# Autodesk Inventor assembly: Cucina
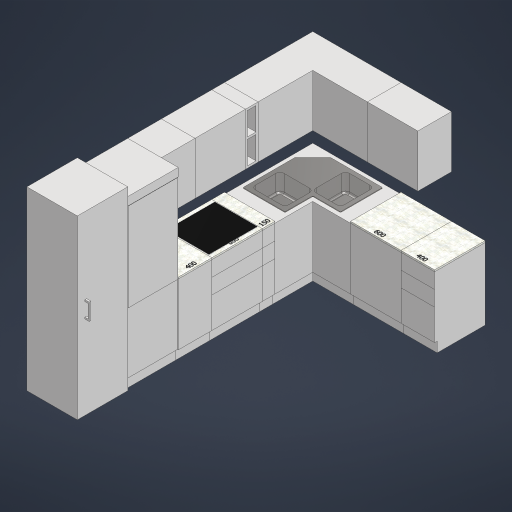
[picture p0: Inventor's stored thumbnail of the model, 512x512]
Saved by Autodesk Inventor 2024.2 (Build 282272000, 272)
## iProperties
Created: 2025-08-27
Part Number: Cucina
Document SubType Name: Assembly
Designer: Luca
Author: Luca
## iProperties of the stored document MemberDocs/xUfgzgntkA0k4y0erJhm34xwdJg
Created: 2025-08-27
Part Number: Cucina
Document SubType Name: Assembly
Designer: Luca
Mass: 4.3593e+06 g
Surface Area: 422535 cm^2
Volume: 4.3593e+06 cm^3
Density: 1 g/cm^3
Author: Luca
## iProperties of the stored document MemberDocs/xWfym0oruPsuzs3vjEgnhmlbwMf
Created: 2025-08-27
Part Number: Cucina
Document SubType Name: Assembly
Designer: Luca
Mass: 4.21038e+06 g
Surface Area: 416936 cm^2
Volume: 4.21038e+06 cm^3
Density: 1 g/cm^3
Author: Luca
## Documents named in this file (10)
- C:\Users\tecnico11\Desktop\Luca\Torre\Cucina.iam
- C:\Users\tecnico11\Desktop\Luca\Torre\Mobile lavandino angolo.ipt
- C:\Users\tecnico11\Desktop\Luca\Torre\Lavandino ad angolo Apell ROAN2IBC.ipt
- C:\Users\tecnico11\Desktop\Luca\Torre\Frigorifero.ipt
- C:\Users\tecnico11\Desktop\Luca\Torre\Mobile cucina.ipt
- C:\Users\tecnico11\Desktop\Luca\Torre\Piano cottura.ipt
- C:\Users\tecnico11\Desktop\Luca\Torre\Pensile.ipt
- C:\Users\tecnico11\Desktop\Luca\Torre\Pensile angolo.ipt
- C:\Users\tecnico11\Desktop\Luca\Torre\Mobile angolo.ipt
- C:\Users\tecnico11\Desktop\Luca\Torre\Mobile lavandino.ipt
## Components (15 placed, 7 different names)
1. Mobile lavandino angolo:1 — Mate:5, Mate:6, Mate:7, Rigid:10, Rigid:13
2. Lavandino ad angolo Apell ROAN2IBC:1
3. Frigorifero:1 — Rigid:11
4. Mobile cucina:1 — Rigid:11
5. Mobile cucina:2 — Rigid:13
6. Mobile cucina:3 — Rigid:10
7. Mobile cucina:4
8. Mobile cucina:5
9. Mobile cucina:6
10. Piano cottura:1
11. Pensile:1
12. Pensile:2 — Rigid:12
13. Pensile:3 — Mate:8, Mate:9
14. Pensile:4 — Mate:10, Mate:11
15. Pensile angolo:1 — Mate:8, Mate:9, Mate:10, Mate:11, Rigid:12
## Relationships (26: WeldJoint 13, Mate 10, Flush 2, Angle 1)
- [Mate]: Mobile lavandino angolo:1 ↔ Lavandino ad angolo Apell ROAN2IBC:1
- [Angle] (180 deg): Mobile lavandino angolo:1 ↔ Lavandino ad angolo Apell ROAN2IBC:1
- [Mate]: Mobile lavandino angolo:1 ↔ Lavandino ad angolo Apell ROAN2IBC:1
- [Mate] (32 mm): Mobile lavandino angolo:1 ↔ Lavandino ad angolo Apell ROAN2IBC:1
- [WeldJoint]: Mobile cucina:2 ↔ Mobile cucina:4
- [WeldJoint]: Mobile cucina:2 ↔ Mobile cucina:3
- [WeldJoint]: Mobile cucina:1 ↔ Mobile cucina:4
- [WeldJoint]: Mobile cucina:5 ↔ Mobile cucina:6
- [WeldJoint]: Mobile lavandino angolo:1 ↔ Mobile cucina:5
- [WeldJoint]: Mobile cucina:2 ↔ Piano cottura:1
- [WeldJoint]: Pensile:1 ↔ Pensile:2
- [WeldJoint]: Mobile cucina:1 ↔ Pensile:1
- [WeldJoint]: Pensile:2 ↔ Pensile:3
- [Flush]: Mobile cucina:5 ↔ Pensile:4
- Mate:5: Mobile lavandino angolo:1
- Mate:6: Mobile lavandino angolo:1
- Mate:7: Mobile lavandino angolo:1
- Rigid:10 [WeldJoint]: Mobile lavandino angolo:1 ↔ Mobile cucina:3
- Rigid:11 [WeldJoint]: Frigorifero:1 ↔ Mobile cucina:1
- Flush:3 (2875 mm)
- Mate:8: Pensile:3 ↔ Pensile angolo:1
- Mate:9: Pensile:3 ↔ Pensile angolo:1
- Mate:10: Pensile:4 ↔ Pensile angolo:1
- Mate:11: Pensile:4 ↔ Pensile angolo:1
- Rigid:12 [WeldJoint]: Pensile:2 ↔ Pensile angolo:1
- Rigid:13 [WeldJoint]: Mobile lavandino angolo:1 ↔ Mobile cucina:2
## Named parameters: d100_d98 = 0 mm
